# Autodesk Inventor assembly: Slider
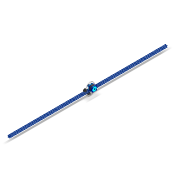
[picture p0: Inventor's stored thumbnail of the model, 180x180]
Saved by Autodesk Inventor 2020 (Build 240168000, 168)
## iProperties
Created: 2020-03-27
Part Number: Slider
Document SubType Name: Assembly
Designer: chitl
Author: chitl
## Documents named in this file (8)
- C:\Users\chitl\Desktop\CNC-Drawing-Robot\Inventor Files\Y-Axis\Slider.iam
- C:\Users\chitl\Desktop\CNC-Drawing-Robot\Inventor Files\Y-Axis\Slider_Wall.ipt
- C:\Users\chitl\Desktop\CNC-Drawing-Robot\Inventor Files\VSlots\V-Slot Rail (20x20x500).ipt
- C:\Users\chitl\Desktop\CNC-Drawing-Robot\Inventor Files\Y-Axis\V_Bearing.iam
- C:\Users\chitl\Desktop\CNC-Drawing-Robot\Inventor Files\Y-Axis\Spacer.ipt
- C:\Users\chitl\Desktop\CNC-Drawing-Robot\Inventor Files\NEMA Motor\NEMA17_GT2B5W10.iam
- C:\Users\chitl\Desktop\CNC-Drawing-Robot\Inventor Files\Fastners\M3-Black-Oxide\91290A117_BLACK-OXIDE CLASS 12.9 SOCKET HEAD CAP SCREW.ipt
- C:\Users\chitl\Desktop\CNC-Drawing-Robot\Inventor Files\Y-Axis\Delrin V-Wheel.ipt
## Components (16 placed, 7 different names)
1. Slider_Wall:1 — Mate:5, Mate:6, Mate:7, Mate:8, Mate:9
2. V-Slot Rail (20x20x500):1
3. V_Bearing:1 [sub-assembly]
4. V_Bearing:2 [sub-assembly]
5. V_Bearing:3 [sub-assembly]
6. Spacer:1 — Mate:4
7. Spacer:2 — Mate:4
8. NEMA17_GT2B5W10:1 [sub-assembly] — Mate:5
9. V-Slot Rail (20x20x500):2
10. Delrin V-Wheel:1
11. Delrin V-Wheel:2
12. Delrin V-Wheel:3
13. 91290A117_BLACK-OXIDE CLASS 12.9 SOCKET HEAD CAP SCREW:4 — Mate:6
14. 91290A117_BLACK-OXIDE CLASS 12.9 SOCKET HEAD CAP SCREW:2 — Mate:8
15. 91290A117_BLACK-OXIDE CLASS 12.9 SOCKET HEAD CAP SCREW:3 — Mate:7
16. 91290A117_BLACK-OXIDE CLASS 12.9 SOCKET HEAD CAP SCREW:1 — Mate:9
## Relationships (6: Mate 6)
- Mate:4: Spacer:1 ↔ Spacer:2
- Mate:5: Slider_Wall:1 ↔ NEMA17_GT2B5W10:1
- Mate:6: Slider_Wall:1 ↔ 91290A117_BLACK-OXIDE CLASS 12.9 SOCKET HEAD CAP SCREW:4
- Mate:7: Slider_Wall:1 ↔ 91290A117_BLACK-OXIDE CLASS 12.9 SOCKET HEAD CAP SCREW:3
- Mate:8: Slider_Wall:1 ↔ 91290A117_BLACK-OXIDE CLASS 12.9 SOCKET HEAD CAP SCREW:2
- Mate:9: Slider_Wall:1 ↔ 91290A117_BLACK-OXIDE CLASS 12.9 SOCKET HEAD CAP SCREW:1
